# Autodesk Inventor assembly: ensamble_general
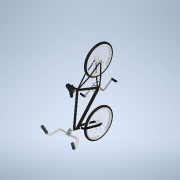
[picture p0: Inventor's stored thumbnail of the model, 180x180]
Saved by Autodesk Inventor 2021 (Build 250183000, 183)
## iProperties
Created: 2021-07-05
Part Number: ensamble_general
Document SubType Name: Assembly
Designer: j2seb
Author: j2seb
## Documents named in this file (11)
- C:\Git\Proyecto_APM\02 Inventor\bicicleta_ruta\ensamble_general.iam
- C:\Git\Proyecto_APM\02 Inventor\bicicleta_ruta\marco_bicicleta.ipt
- C:\Git\Proyecto_APM\02 Inventor\bicicleta_ruta\Manubrio\Manubrio.iam
- C:\Git\Proyecto_APM\02 Inventor\bicicleta_ruta\sillin.iam
- C:\Git\Proyecto_APM\02 Inventor\bicicleta_ruta\otros\caja_pedalera.iam
- C:\Git\Proyecto_APM\02 Inventor\bicicleta_ruta\otros\llanta delantera.iam
- C:\Git\Proyecto_APM\02 Inventor\bicicleta_ruta\otros\llanta trasera.iam
- C:\Git\Proyecto_APM\02 Inventor\bicicleta_ruta\otros\cubrecadena.ipt
- C:\Git\Proyecto_APM\02 Inventor\bicicleta_ruta\otros\lamina_eje_trasero.ipt
- C:\Git\Proyecto_APM\02 Inventor\bicicleta_ruta\Transmision\Cadena.iam
- C:\Git\Proyecto_APM\02 Inventor\bicicleta_ruta\otros\ajuste_silin.ipt
## Components (11 placed, 10 different names)
1. marco_bicicleta:1 — Mate:1, Mate:2, Mate:3, Mate:4, Mate:5, Mate:6, Mate:7, Mate:8, Mate:10, Mate:12, Mate:23
2. Manubrio:1 [sub-assembly] — Mate:1, Mate:9
3. sillin:1 [sub-assembly] — Mate:2
4. caja_pedalera:1 [sub-assembly] — Mate:3, Mate:4, Mate:21, Mate:22
5. llanta trasera:1 [sub-assembly] — Mate:13, Mate:14, Mate:17, Mate:18, Mate:19, Mate:20
6. llanta delantera:1 [sub-assembly] — Mate:15, Mate:16
7. cubrecadena:1 — Mate:21
8. lamina_eje_trasero:1 — Mate:19, Mate:20
9. lamina_eje_trasero:2 — Mate:17, Mate:18
10. Cadena:1 [sub-assembly] — Mate:22
11. ajuste_silin:1 — Mate:23
## Relationships (25: Mate 22, Angle 3)
- Mate:1: marco_bicicleta:1 ↔ Manubrio:1
- Mate:2: marco_bicicleta:1 ↔ sillin:1
- Mate:3: marco_bicicleta:1 ↔ caja_pedalera:1
- Mate:4: marco_bicicleta:1 ↔ caja_pedalera:1
- Mate:5: marco_bicicleta:1
- Angle:1 (0 deg)
- Mate:6: marco_bicicleta:1
- Mate:7: marco_bicicleta:1
- Mate:8: marco_bicicleta:1
- Mate:9: Manubrio:1
- Mate:10: marco_bicicleta:1
- Angle:2 (0 deg)
- Mate:12: marco_bicicleta:1
- Angle:3 (0 deg)
- Mate:13: llanta trasera:1
- Mate:14: llanta trasera:1
- Mate:15: llanta delantera:1
- Mate:16: llanta delantera:1
- Mate:17: llanta trasera:1 ↔ lamina_eje_trasero:2
- Mate:18: llanta trasera:1 ↔ lamina_eje_trasero:2
- Mate:19: llanta trasera:1 ↔ lamina_eje_trasero:1
- Mate:20: llanta trasera:1 ↔ lamina_eje_trasero:1
- Mate:21: caja_pedalera:1 ↔ cubrecadena:1
- Mate:22: caja_pedalera:1 ↔ Cadena:1
- Mate:23: marco_bicicleta:1 ↔ ajuste_silin:1
